# Autodesk Inventor assembly: DriveWheelAssembly_MIR
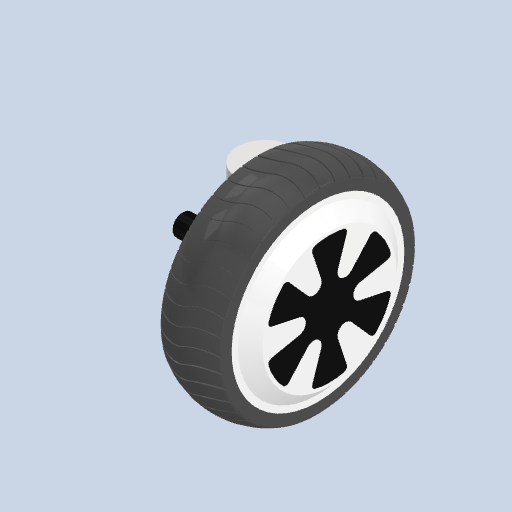
[picture p0: Inventor's stored thumbnail of the model, 512x512]
Saved by Autodesk Inventor 2023 (Build 270158000, 158)
## iProperties
Created: 2022-12-26
Part Number: DriveWheelAssembly_MIR
Document SubType Name: Assembly
Designer: haash
Author: haash
## Documents named in this file (8)
- C:\Users\haash\OneDrive\Documents\Projects\Hoverboard-Robot\DriveWheelAssembly_MIR.iam
- C:\Users\haash\OneDrive\Documents\Projects\Hoverboard-Robot\Hoverboard-Wheel\Motor, BLDC, Hoverboard Wheel, 6.5in_MIR.ipt
- C:\Users\haash\OneDrive\Documents\Projects\Hoverboard-Robot\Hoverboard Frame_MIR.ipt
- C:\Users\haash\OneDrive\Documents\Projects\Hoverboard-Robot\EncoderTimingBelt_MIR.ipt
- C:\Users\haash\OneDrive\Documents\Projects\Hoverboard-Robot\EncoderPully_MIR.ipt
- C:\Users\haash\OneDrive\Documents\Projects\Hoverboard-Robot\WheelPully_MIR.ipt
- C:\Users\haash\OneDrive\Documents\Projects\Hoverboard-Robot\EncoderMount_MIR.ipt
- C:\Users\haash\OneDrive\Documents\Projects\Hoverboard-Robot\Encoder\38 mm OD, 6 mm Shaft, Incremental Optical Rotary Encoder_MIR.iam
## Components (7 placed, 7 different names)
1. Motor, BLDC, Hoverboard Wheel, 6.5in_MIR:1 — Mate:2, Mate:9, Mate:1
2. Hoverboard Frame_MIR:1 — Mate:3, Mate:5, Mate:4
3. EncoderTimingBelt_MIR:1 — Mate:2, Mate:11, Mate:12
4. EncoderPully_MIR:1 — Mate:11, Mate:8, Mate:10
5. WheelPully_MIR:1 — Mate:9, Mate:12, Mate:1, Mate:8
6. EncoderMount_MIR:1 — Mate:3, Mate:5, Mate:4, Mate:7, Mate:6, Angle:1
7. 38 mm OD, 6 mm Shaft, Incremental Optical Rotary Encoder_MIR:1 [sub-assembly] — Mate:10, Mate:7, Mate:6, Angle:1
## Relationships (13: Mate 12, Angle 1)
- Mate:2: Motor, BLDC, Hoverboard Wheel, 6.5in_MIR:1 ↔ EncoderTimingBelt_MIR:1
- Mate:11: EncoderTimingBelt_MIR:1 ↔ EncoderPully_MIR:1
- Mate:9: Motor, BLDC, Hoverboard Wheel, 6.5in_MIR:1 ↔ WheelPully_MIR:1
- Mate:12: EncoderTimingBelt_MIR:1 ↔ WheelPully_MIR:1
- Mate:1: Motor, BLDC, Hoverboard Wheel, 6.5in_MIR:1 ↔ WheelPully_MIR:1
- Mate:8: EncoderPully_MIR:1 ↔ WheelPully_MIR:1
- Mate:3: Hoverboard Frame_MIR:1 ↔ EncoderMount_MIR:1
- Mate:5: Hoverboard Frame_MIR:1 ↔ EncoderMount_MIR:1
- Mate:4: Hoverboard Frame_MIR:1 ↔ EncoderMount_MIR:1
- Mate:10: EncoderPully_MIR:1 ↔ 38 mm OD, 6 mm Shaft, Incremental Optical Rotary Encoder_MIR:1
- Mate:7: EncoderMount_MIR:1 ↔ 38 mm OD, 6 mm Shaft, Incremental Optical Rotary Encoder_MIR:1
- Mate:6: EncoderMount_MIR:1 ↔ 38 mm OD, 6 mm Shaft, Incremental Optical Rotary Encoder_MIR:1
- Angle:1 (0 deg): EncoderMount_MIR:1 ↔ 38 mm OD, 6 mm Shaft, Incremental Optical Rotary Encoder_MIR:1
